# Autodesk Inventor assembly: Assembly - GantryPlate
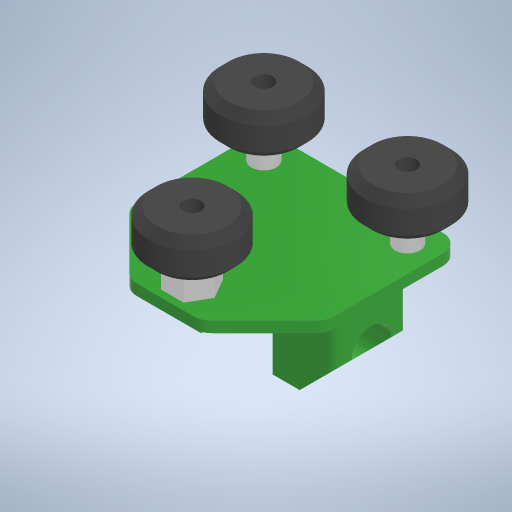
[picture p0: Inventor's stored thumbnail of the model, 512x512]
Saved by Autodesk Inventor 2023 (Build 270158000, 158)
## iProperties
Created: 2023-04-10
Part Number: Assembly - GantryPlate
Document SubType Name: Assembly
Designer: ethan
Author: ethan
## Documents named in this file (5)
- D:\Documents\GitHub\WU-AutomaticChessboard\CAD\Assembly - GantryPlate.iam
- D:\Documents\GitHub\WU-AutomaticChessboard\CAD\EccentricNut 5mmID 11mmHex.ipt
- D:\Documents\GitHub\WU-AutomaticChessboard\CAD\Gantry Plate - Sides.ipt
- D:\Documents\GitHub\WU-AutomaticChessboard\CAD\VSlot RollerWheel.ipt
- D:\Documents\GitHub\WU-AutomaticChessboard\CAD\Spacer 5mmID 8mmOD.ipt
## Components (7 placed, 4 different names)
1. EccentricNut 5mmID 11mmHex:1 — Rigid:1, Rotational:8
2. Gantry Plate - Sides:1 — Rigid:1, Rigid:2, Rigid:3
3. VSlot RollerWheel:1 — Rotational:7
4. VSlot RollerWheel:2 — Rotational:6
5. VSlot RollerWheel:3 — Rotational:8
6. Spacer 5mmID 8mmOD:1 — Rigid:2, Rotational:7
7. Spacer 5mmID 8mmOD:2 — Rigid:3, Rotational:6
## Relationships (6: WeldJoint 3, RevoluteJoint 3)
- Rigid:1 [WeldJoint]: EccentricNut 5mmID 11mmHex:1 ↔ Gantry Plate - Sides:1
- Rigid:2 [WeldJoint]: Gantry Plate - Sides:1 ↔ Spacer 5mmID 8mmOD:1
- Rigid:3 [WeldJoint]: Gantry Plate - Sides:1 ↔ Spacer 5mmID 8mmOD:2
- Rotational:7 [RevoluteJoint]: VSlot RollerWheel:1 ↔ Spacer 5mmID 8mmOD:1
- Rotational:6 [RevoluteJoint]: VSlot RollerWheel:2 ↔ Spacer 5mmID 8mmOD:2
- Rotational:8 [RevoluteJoint] (-10 mm): EccentricNut 5mmID 11mmHex:1 ↔ VSlot RollerWheel:3
